# Autodesk Inventor assembly: SSR-40 DA
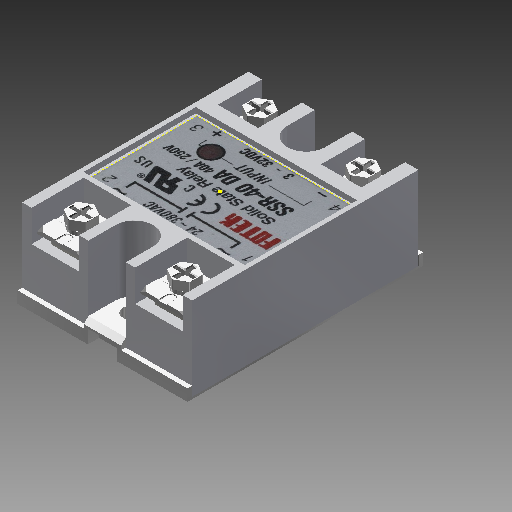
[picture p0: Inventor's stored thumbnail of the model, 512x512]
Saved by Autodesk Inventor 2019 (Build 230136000, 136)
## iProperties
Created: 2014-10-30
Part Number: SSR-40 DA
Document SubType Name: Assembly
Designer: Tyler
Author: Tyler
## Documents named in this file (5)
- C:\Users\Ax\Google Drive\Inventor\Library\SSR-40 DA.iam
- C:\Users\Ax\Google Drive\Inventor\Library\SSR-40 DA BOTTOM.ipt
- C:\Users\Ax\Google Drive\Inventor\Library\SSR-40 DA TOP.ipt
- C:\Users\Ax\Google Drive\Inventor\Library\SSR-40 DA Large P W S.iam
- C:\Users\Ax\Google Drive\Inventor\Library\SSR-40 DA Small P W S.iam
## Components (6 placed, 4 different names)
1. SSR-40 DA BOTTOM:1 — Mate:1, Mate:2
2. SSR-40 DA TOP:1 — Mate:1, Mate:2, Mate:3, Mate:4, Mate:5, Mate:6
3. SSR-40 DA Large P W S:1 [sub-assembly] — Mate:3
4. SSR-40 DA Large P W S:2 [sub-assembly] — Mate:4
5. SSR-40 DA Small P W S:1 [sub-assembly] — Mate:6
6. SSR-40 DA Small P W S:2 [sub-assembly] — Mate:5
## Relationships (6: Mate 6)
- Mate:1: SSR-40 DA BOTTOM:1 ↔ SSR-40 DA TOP:1
- Mate:2: SSR-40 DA BOTTOM:1 ↔ SSR-40 DA TOP:1
- Mate:3: SSR-40 DA TOP:1 ↔ SSR-40 DA Large P W S:1
- Mate:4: SSR-40 DA TOP:1 ↔ SSR-40 DA Large P W S:2
- Mate:5: SSR-40 DA TOP:1 ↔ SSR-40 DA Small P W S:2
- Mate:6: SSR-40 DA TOP:1 ↔ SSR-40 DA Small P W S:1
